# Autodesk Inventor assembly: Motor
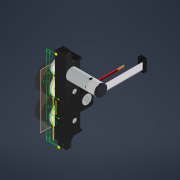
[picture p0: Inventor's stored thumbnail of the model, 180x180]
Saved by Autodesk Inventor 2022 (Build 260153000, 153)
## iProperties
Created: 2021-09-24
Part Number: Motor
Document SubType Name: Assembly
Designer: shiok
Mass: 24.8351 g
Surface Area: 226.347 cm^2
Volume: 18.047 cm^3
Density: 1.37613 g/cm^3
Author: shiok
## Documents named in this file (8)
- C:\Users\shiok\Documents\GitHub\murakumo\inventor\Motor.iam
- C:\Users\shiok\Documents\GitHub\murakumo\inventor\MotorBracket.ipt
- C:\Users\shiok\Documents\GitHub\murakumo\inventor\maxon DCX 10L.iam
- C:\Users\shiok\Documents\GitHub\murakumo\inventor\Tire.iam
- C:\Users\shiok\Documents\GitHub\murakumo\inventor\FL674ZZ.ipt
- C:\Users\shiok\Documents\GitHub\murakumo\inventor\piniongear_41_middle.ipt
- C:\Users\shiok\Documents\GitHub\murakumo\inventor\piniongear_41_src.ipt
- C:\Users\shiok\Documents\GitHub\murakumo\inventor\shaft_short.ipt
## Components (9 placed, 7 different names)
1. MotorBracket:1 — メイト:1, メイト:2, メイト:3, メイト:4, メイト:5, フラッシュ:1, フラッシュ:2, メイト:6, メイト:7, フラッシュ:3, フラッシュ:4, メイト:13, メイト:14, フラッシュ:9
2. maxon DCX 10L:1 [sub-assembly] — メイト:7, メイト:12, メイト:13, メイト:14
3. Tire:1 [sub-assembly] — メイト:5, フラッシュ:1, フラッシュ:4, フラッシュ:7, 対称度:1, フラッシュ:9
4. Tire:2 [sub-assembly] — フラッシュ:2, メイト:6, フラッシュ:3, 対称度:1, メイト:15
5. FL674ZZ:1 — メイト:3, メイト:4, フラッシュ:8
6. FL674ZZ:2 — メイト:1, メイト:2, メイト:16
7. piniongear_41_middle:1 — 挿入:1, メイト:15
8. piniongear_41_src:1 — メイト:12, フラッシュ:7
9. shaft_short:1 — 挿入:1, フラッシュ:8, メイト:16
## Relationships (21: Mate 12, Flush 7, Symmetry 1, Insert 1)
- メイト:1 [Mate]: MotorBracket:1 ↔ FL674ZZ:2
- メイト:2 [Mate]: MotorBracket:1 ↔ FL674ZZ:2
- メイト:3 [Mate]: MotorBracket:1 ↔ FL674ZZ:1
- メイト:4 [Mate]: MotorBracket:1 ↔ FL674ZZ:1
- メイト:5 [Mate]: MotorBracket:1 ↔ Tire:1
- フラッシュ:1 [Flush]: MotorBracket:1 ↔ Tire:1
- フラッシュ:2 [Flush]: MotorBracket:1 ↔ Tire:2
- メイト:6 [Mate]: MotorBracket:1 ↔ Tire:2
- メイト:7 [Mate]: MotorBracket:1 ↔ maxon DCX 10L:1
- フラッシュ:3 [Flush]: MotorBracket:1 ↔ Tire:2
- フラッシュ:4 [Flush]: MotorBracket:1 ↔ Tire:1
- メイト:12 [Mate]: maxon DCX 10L:1 ↔ piniongear_41_src:1
- フラッシュ:7 [Flush]: Tire:1 ↔ piniongear_41_src:1
- メイト:13 [Mate]: MotorBracket:1 ↔ maxon DCX 10L:1
- メイト:14 [Mate]: MotorBracket:1 ↔ maxon DCX 10L:1
- 対称度:1 [Symmetry]: Tire:1 ↔ Tire:2
- 挿入:1 [Insert]: piniongear_41_middle:1 ↔ shaft_short:1
- フラッシュ:8 [Flush]: FL674ZZ:1 ↔ shaft_short:1
- メイト:15 [Mate]: Tire:2 ↔ piniongear_41_middle:1
- メイト:16 [Mate]: FL674ZZ:2 ↔ shaft_short:1
- フラッシュ:9 [Flush]: MotorBracket:1 ↔ Tire:1
